# Autodesk Inventor assembly: Ensamblaje FINAL V1
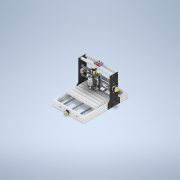
[picture p0: Inventor's stored thumbnail of the model, 180x180]
Saved by Autodesk Inventor 2021 (Build 250183000, 183)
## iProperties
Company: IMT
Created: 2022-05-28
Part Number: Ensamblaje FINAL V1
Document SubType Name: Assembly
Designer: BRAYAN GERSON DURAN TOCONAS
Project: CNC ROUTER IMT 212 P1
Author: BRAYAN GERSON DURAN TOCONAS
Title: CNC
Subject: proyecto IMT 212 P1
Comments: En esta carpeta esta todo el diseño en Inventor y calculos para la construcción de una maquina CNC fresadora para el proyecto final de la materia de diseño de maquinas. Esta CNC es capaz de desplazarse en 3 ejes. 2 por la herramienta y 1 por la base. Además de soportar el torque generador por la herramienta a la hora de gastar el material.
Revision Number: 3
## Documents named in this file (24)
- C:\Users\79449\Documents\CNC_DISENO_DE MAQUINAS\Piezas-Ensambles_Inventor\Ensamblaje FINAL V1.iam
- C:\Users\79449\Documents\CNC_DISENO_DE MAQUINAS\Piezas-Ensambles_Inventor\Primera_presentación\Ensamblaje1.iam
- C:\Users\79449\Documents\CNC_DISENO_DE MAQUINAS\Piezas-Ensambles_Inventor\Segunda_presentación\PlanchaLateral.ipt
- C:\Users\79449\Documents\CNC_DISENO_DE MAQUINAS\Piezas-Ensambles_Inventor\Segunda_presentación\V-SLOT_2020.ipt
- C:\Users\79449\Documents\CNC_DISENO_DE MAQUINAS\Piezas-Ensambles_Inventor\Segunda_presentación\SFU1605-1610\SFU1605 Assem.iam
- C:\Users\79449\Documents\CNC_DISENO_DE MAQUINAS\Piezas-Ensambles_Inventor\Segunda_presentación\Lap rap truc Y.iam
- C:\Users\79449\Documents\CNC_DISENO_DE MAQUINAS\Piezas-Ensambles_Inventor\Segunda_presentación\EjeBase v2.ipt
- C:\Users\79449\Documents\CNC_DISENO_DE MAQUINAS\Piezas-Ensambles_Inventor\Segunda_presentación\De truc Z.iam
- C:\Users\79449\Documents\CNC_DISENO_DE MAQUINAS\Piezas-Ensambles_Inventor\Segunda_presentación\ImpresionSoporte.ipt
- C:\Users\79449\Documents\CNC_DISENO_DE MAQUINAS\Piezas-Ensambles_Inventor\Segunda_presentación\Kep Truc KLF-10.ipt
- C:\Users\79449\Documents\CNC_DISENO_DE MAQUINAS\Piezas-Ensambles_Inventor\Segunda_presentación\Nema17\Assembly1.iam
- C:\Users\79449\Documents\CNC_DISENO_DE MAQUINAS\Piezas-Ensambles_Inventor\Segunda_presentación\Flexible Coupling 10-5.ipt
- C:\Users\79449\Documents\CNC_DISENO_DE MAQUINAS\Piezas-Ensambles_Inventor\Segunda_presentación\KFL003 block flange ball bearing 17 diameter shaft.ipt
- C:\Users\79449\Documents\Inventor\Content Center Files\R2021\es-ES\ANSI_ASME B18.5\ANSI_ASME B18.5 - 1_4 - 20 - 1 - 1_4-20 UNC.ipt
- C:\Users\79449\Documents\Inventor\Content Center Files\R2021\es-ES\BS 4183(1)\BS 4183 - M6(1).ipt
- C:\Users\79449\Documents\Inventor\Content Center Files\R2021\es-ES\AS 1110\AS 1110 - M4 x 25.ipt
- C:\Users\79449\Documents\Inventor\Content Center Files\R2021\es-ES\AS 1110\AS 1110 - M2,5 x 20.ipt
- C:\Users\79449\Documents\Inventor\Content Center Files\R2021\es-ES\AS 1110\AS 1110 - M2,5 x 10.ipt
- C:\Users\79449\Documents\Inventor\Content Center Files\R2021\es-ES\U 3284(2)\Unbrako. Hallowell Steel Collars. Inch Series - 0.5 x 1 x 7_16.ipt
- C:\Users\79449\Documents\Inventor\Content Center Files\R2021\es-ES\BS EN 24017\ISO 4017 - M4 x 8BS EN.ipt
- C:\Users\79449\Documents\Inventor\Content Center Files\R2021\es-ES\AS 1112 (2)\AS 1112 - M4  Tipo 5.ipt
- C:\Users\79449\Documents\Inventor\Content Center Files\R2021\es-ES\AS 1110\AS 1110 - M4 x 20.ipt
- C:\Users\79449\Documents\CNC_DISENO_DE MAQUINAS\Piezas-Ensambles_Inventor\Segunda_presentación\Arduino_CNC_Assembly.ipt
- C:\Users\79449\Documents\Inventor\Content Center Files\R2021\es-ES\AS 1112 (2)\AS 1112 - M2,5  Tipo 5.ipt
## Components (75 placed, 23 different names)
1. Ensamblaje1:1 [sub-assembly] — Nivelación:1, Coincidencia:1, Nivelación:2, Coincidencia:2, Nivelación:4, Coincidencia:23, Nivelación:13, Nivelación:14, Nivelación:15, Coincidencia:44, Coincidencia:45, Coincidencia:49, Coincidencia:50, Coincidencia:52, Coincidencia:54
2. PlanchaLateral:2 — Coincidencia:2, Nivelación:4, Coincidencia:13, Nivelación:8, Coincidencia:15, Coincidencia:19, Nivelación:11, Coincidencia:20, Nivelación:12, Nivelación:15, Coincidencia:24, Nivelación:20, Coincidencia:37, Coincidencia:39, Coincidencia:40, Coincidencia:73, Coincidencia:74, Coincidencia:75, Coincidencia:76, Coincidencia:85, Coincidencia:86, Coincidencia:87, Coincidencia:88, Coincidencia:93, Coincidencia:94, Coincidencia:113, Coincidencia:114, Coincidencia:115, Coincidencia:116, Coincidencia:117, Coincidencia:118, Coincidencia:119, Coincidencia:120, Coincidencia:121, Coincidencia:122, Coincidencia:123, Coincidencia:124, Coincidencia:125, Coincidencia:126, Coincidencia:127, Coincidencia:128, Coincidencia:130, Coincidencia:132, Coincidencia:134, Coincidencia:136, Coincidencia:138, Coincidencia:140, Coincidencia:154, Coincidencia:156, Coincidencia:158, Coincidencia:166
3. V-SLOT_2020:2 — Coincidencia:13, Coincidencia:16, Nivelación:16, Nivelación:17, Coincidencia:155, Coincidencia:159, Coincidencia:165, Nivelación:21
4. SFU1605 Assem:1 [sub-assembly] — Coincidencia:14, Coincidencia:38, Coincidencia:41, Coincidencia:43
5. Lap rap truc Y:1 [sub-assembly] — Coincidencia:14, Ángulo:1, Coincidencia:18, Coincidencia:21, Coincidencia:22, Coincidencia:27, Coincidencia:28, Coincidencia:29, Coincidencia:30
6. V-SLOT_2020:3 — Nivelación:8, Coincidencia:15, Coincidencia:16, Nivelación:19, Nivelación:20, Coincidencia:157, Coincidencia:163
7. V-SLOT_2020:4 — Coincidencia:18, Nivelación:18, Coincidencia:153, Coincidencia:161
8. EjeBase v2:1 — Coincidencia:19, Nivelación:11, Coincidencia:24, Coincidencia:25, Coincidencia:27, Coincidencia:28, Coincidencia:89, Coincidencia:91
9. EjeBase v2:2 — Coincidencia:20, Nivelación:12, Coincidencia:26, Coincidencia:29, Coincidencia:30, Coincidencia:90, Coincidencia:92
10. De truc Z:1 [sub-assembly] — Coincidencia:21, Coincidencia:22
11. PlanchaLateral:3 — Coincidencia:23, Nivelación:13, Nivelación:14, Nivelación:16, Nivelación:17, Nivelación:18, Coincidencia:25, Coincidencia:26, Nivelación:19, Coincidencia:31, Coincidencia:32, Coincidencia:33, Coincidencia:62, Coincidencia:64, Coincidencia:66, Coincidencia:68, Coincidencia:70, Coincidencia:72, Coincidencia:95, Coincidencia:96, Coincidencia:97, Coincidencia:98, Coincidencia:99, Coincidencia:100, Coincidencia:101, Coincidencia:102, Coincidencia:103, Coincidencia:104, Coincidencia:105, Coincidencia:106, Coincidencia:107, Coincidencia:108, Coincidencia:109, Coincidencia:110, Coincidencia:111, Coincidencia:112, Coincidencia:142, Coincidencia:144, Coincidencia:146, Coincidencia:148, Coincidencia:150, Coincidencia:152, Coincidencia:160, Coincidencia:162, Coincidencia:164
12. ImpresionSoporte:1 — Coincidencia:31, Coincidencia:32, Coincidencia:33, Coincidencia:34, Coincidencia:35, Coincidencia:36, Coincidencia:65, Coincidencia:67, Coincidencia:69, Coincidencia:71, Coincidencia:168, Coincidencia:170, Coincidencia:172, Coincidencia:174
13. Kep Truc KLF-10:1 — Coincidencia:34, Coincidencia:35, Coincidencia:36, Coincidencia:61, Coincidencia:63, Coincidencia:176, Coincidencia:178
14. Assembly1:1 [sub-assembly] — Coincidencia:37, Coincidencia:38, Coincidencia:39, Coincidencia:40, Coincidencia:42
15. Flexible Coupling 10-5:1 — Coincidencia:41, Coincidencia:42, Coincidencia:43
16. KFL003 block flange ball bearing 17 diameter shaft:1 — Coincidencia:44, Coincidencia:45, Coincidencia:51, Coincidencia:53, Coincidencia:58, Coincidencia:60
17. Perno de cabeza en T - Pulgadas 1/4 - 20 - 1:1 — Coincidencia:49, Coincidencia:50, Coincidencia:51, Coincidencia:57
18. Perno de cabeza en T - Pulgadas 1/4 - 20 - 1:2 — Coincidencia:52, Coincidencia:53, Coincidencia:54, Coincidencia:59
19. BS 4183 - Métrico M6:2 — Coincidencia:57, Coincidencia:58
20. BS 4183 - Métrico M6:3 — Coincidencia:59, Coincidencia:60
21. AS 1110 - Métrico M4 x 25:1 — Coincidencia:61, Coincidencia:62, Coincidencia:175
22. AS 1110 - Métrico M4 x 25:2 — Coincidencia:63, Coincidencia:64, Coincidencia:177
23. AS 1110 - Métrico M2,5 x 20:1 — Coincidencia:65, Coincidencia:66, Coincidencia:167
24. AS 1110 - Métrico M2,5 x 20:2 — Coincidencia:67, Coincidencia:68, Coincidencia:173
25. AS 1110 - Métrico M2,5 x 20:3 — Coincidencia:69, Coincidencia:70, Coincidencia:169
26. AS 1110 - Métrico M2,5 x 20:4 — Coincidencia:71, Coincidencia:72, Coincidencia:171
27. AS 1110 - Métrico M2,5 x 10:1 — Coincidencia:73, Coincidencia:74
28. AS 1110 - Métrico M2,5 x 10:2 — Coincidencia:75, Coincidencia:76
29. AS 1110 - Métrico M2,5 x 10:7 — Coincidencia:85, Coincidencia:86
30. AS 1110 - Métrico M2,5 x 10:8 — Coincidencia:87, Coincidencia:88
31. Anillo de ajuste 0.5 x 1 x 7/16:1 — Coincidencia:90, Coincidencia:96
32. Anillo de ajuste 0.5 x 1 x 7/16:2 — Coincidencia:89, Coincidencia:95
33. Anillo de ajuste 0.5 x 1 x 7/16:3 — Coincidencia:91, Coincidencia:93
34. Anillo de ajuste 0.5 x 1 x 7/16:4 — Coincidencia:92, Coincidencia:94
35. BS EN 24017 - Métrico M4 x 8:1 — Coincidencia:97, Coincidencia:98, Coincidencia:151
36. BS EN 24017 - Métrico M4 x 8:2 — Coincidencia:99, Coincidencia:100
37. BS EN 24017 - Métrico M4 x 8:3 — Coincidencia:101, Coincidencia:102
38. BS EN 24017 - Métrico M4 x 8:4 — Coincidencia:103, Coincidencia:104, Coincidencia:143
39. BS EN 24017 - Métrico M4 x 8:5 — Coincidencia:105, Coincidencia:106, Coincidencia:141
40. BS EN 24017 - Métrico M4 x 8:6 — Coincidencia:107, Coincidencia:108, Coincidencia:147
41. BS EN 24017 - Métrico M4 x 8:7 — Coincidencia:109, Coincidencia:110, Coincidencia:149
42. BS EN 24017 - Métrico M4 x 8:8 — Coincidencia:111, Coincidencia:112, Coincidencia:145
43. BS EN 24017 - Métrico M4 x 8:9 — Coincidencia:113, Coincidencia:114, Coincidencia:137
44. BS EN 24017 - Métrico M4 x 8:10 — Coincidencia:115, Coincidencia:116
45. BS EN 24017 - Métrico M4 x 8:11 — Coincidencia:117, Coincidencia:118
46. BS EN 24017 - Métrico M4 x 8:12 — Coincidencia:119, Coincidencia:120, Coincidencia:129
47. BS EN 24017 - Métrico M4 x 8:13 — Coincidencia:121, Coincidencia:122, Coincidencia:135
48. BS EN 24017 - Métrico M4 x 8:14 — Coincidencia:123, Coincidencia:124, Coincidencia:133
49. BS EN 24017 - Métrico M4 x 8:15 — Coincidencia:125, Coincidencia:126, Coincidencia:131
50. BS EN 24017 - Métrico M4 x 8:16 — Coincidencia:127, Coincidencia:128, Coincidencia:139
51. AS 1112 (2) - Métrico M4  Tipo 5:1 — Coincidencia:129, Coincidencia:130
52. AS 1112 (2) - Métrico M4  Tipo 5:2 — Coincidencia:131, Coincidencia:132
53. AS 1112 (2) - Métrico M4  Tipo 5:3 — Coincidencia:133, Coincidencia:134
54. AS 1112 (2) - Métrico M4  Tipo 5:4 — Coincidencia:135, Coincidencia:136
55. AS 1112 (2) - Métrico M4  Tipo 5:5 — Coincidencia:137, Coincidencia:138
56. AS 1112 (2) - Métrico M4  Tipo 5:6 — Coincidencia:139, Coincidencia:140
57. AS 1112 (2) - Métrico M4  Tipo 5:7 — Coincidencia:141, Coincidencia:142
58. AS 1112 (2) - Métrico M4  Tipo 5:8 — Coincidencia:143, Coincidencia:144
59. AS 1112 (2) - Métrico M4  Tipo 5:9 — Coincidencia:145, Coincidencia:146
60. AS 1112 (2) - Métrico M4  Tipo 5:10 — Coincidencia:147, Coincidencia:148
61. AS 1112 (2) - Métrico M4  Tipo 5:11 — Coincidencia:149, Coincidencia:150
62. AS 1112 (2) - Métrico M4  Tipo 5:12 — Coincidencia:151, Coincidencia:152
63. AS 1110 - Métrico M4 x 20:1 — Coincidencia:153, Coincidencia:154
64. AS 1110 - Métrico M4 x 20:2 — Coincidencia:155, Coincidencia:156
65. AS 1110 - Métrico M4 x 20:3 — Coincidencia:157, Coincidencia:158
66. AS 1110 - Métrico M4 x 20:4 — Coincidencia:159, Coincidencia:160
67. AS 1110 - Métrico M4 x 20:5 — Coincidencia:161, Coincidencia:162
68. AS 1110 - Métrico M4 x 20:6 — Coincidencia:163, Coincidencia:164
69. Arduino_CNC_Assembly:1 — Coincidencia:165, Nivelación:21, Coincidencia:166
70. AS 1112 (2) - Métrico M2,5  Tipo 5:1 — Coincidencia:167, Coincidencia:168
71. AS 1112 (2) - Métrico M2,5  Tipo 5:2 — Coincidencia:169, Coincidencia:170
72. AS 1112 (2) - Métrico M2,5  Tipo 5:3 — Coincidencia:171, Coincidencia:172
73. AS 1112 (2) - Métrico M2,5  Tipo 5:4 — Coincidencia:173, Coincidencia:174
74. AS 1112 (2) - Métrico M4  Tipo 5:13 — Coincidencia:175, Coincidencia:176
75. AS 1112 (2) - Métrico M4  Tipo 5:14 — Coincidencia:177, Coincidencia:178
## Relationships (170: Mate 154, Flush 15, Angle 1)
- Nivelación:1 [Flush]: Ensamblaje1:1
- Coincidencia:1 [Mate]: Ensamblaje1:1
- Nivelación:2 [Flush]: Ensamblaje1:1
- Coincidencia:2 [Mate]: Ensamblaje1:1 ↔ PlanchaLateral:2
- Nivelación:4 [Flush]: Ensamblaje1:1 ↔ PlanchaLateral:2
- Coincidencia:13 [Mate]: PlanchaLateral:2 ↔ V-SLOT_2020:2
- Coincidencia:14 [Mate]: SFU1605 Assem:1 ↔ Lap rap truc Y:1
- Ángulo:1 [Angle] (0 deg): Lap rap truc Y:1
- Nivelación:8 [Flush]: PlanchaLateral:2 ↔ V-SLOT_2020:3
- Coincidencia:15 [Mate]: PlanchaLateral:2 ↔ V-SLOT_2020:3
- Coincidencia:16 [Mate] (130 mm): V-SLOT_2020:2 ↔ V-SLOT_2020:3
- Coincidencia:18 [Mate]: Lap rap truc Y:1 ↔ V-SLOT_2020:4
- Coincidencia:19 [Mate]: PlanchaLateral:2 ↔ EjeBase v2:1
- Nivelación:11 [Flush]: PlanchaLateral:2 ↔ EjeBase v2:1
- Coincidencia:20 [Mate]: PlanchaLateral:2 ↔ EjeBase v2:2
- Nivelación:12 [Flush]: PlanchaLateral:2 ↔ EjeBase v2:2
- Coincidencia:21 [Mate]: Lap rap truc Y:1 ↔ De truc Z:1
- Coincidencia:22 [Mate]: Lap rap truc Y:1 ↔ De truc Z:1
- Coincidencia:23 [Mate]: Ensamblaje1:1 ↔ PlanchaLateral:3
- Nivelación:13 [Flush]: Ensamblaje1:1 ↔ PlanchaLateral:3
- Nivelación:14 [Flush] (100 mm): Ensamblaje1:1 ↔ PlanchaLateral:3
- Nivelación:15 [Flush] (-100 mm): Ensamblaje1:1 ↔ PlanchaLateral:2
- Nivelación:16 [Flush]: V-SLOT_2020:2 ↔ PlanchaLateral:3
- Nivelación:17 [Flush]: V-SLOT_2020:2 ↔ PlanchaLateral:3
- Nivelación:18 [Flush]: V-SLOT_2020:4 ↔ PlanchaLateral:3
- Coincidencia:24 [Mate]: PlanchaLateral:2 ↔ EjeBase v2:1
- Coincidencia:25 [Mate]: EjeBase v2:1 ↔ PlanchaLateral:3
- Coincidencia:26 [Mate]: EjeBase v2:2 ↔ PlanchaLateral:3
- Nivelación:19 [Flush]: V-SLOT_2020:3 ↔ PlanchaLateral:3
- Nivelación:20 [Flush]: PlanchaLateral:2 ↔ V-SLOT_2020:3
- Coincidencia:27 [Mate]: Lap rap truc Y:1 ↔ EjeBase v2:1
- Coincidencia:28 [Mate]: Lap rap truc Y:1 ↔ EjeBase v2:1
- Coincidencia:29 [Mate]: Lap rap truc Y:1 ↔ EjeBase v2:2
- Coincidencia:30 [Mate]: Lap rap truc Y:1 ↔ EjeBase v2:2
- Coincidencia:31 [Mate]: PlanchaLateral:3 ↔ ImpresionSoporte:1
- Coincidencia:32 [Mate]: PlanchaLateral:3 ↔ ImpresionSoporte:1
- Coincidencia:33 [Mate]: PlanchaLateral:3 ↔ ImpresionSoporte:1
- Coincidencia:34 [Mate]: ImpresionSoporte:1 ↔ Kep Truc KLF-10:1
- Coincidencia:35 [Mate]: ImpresionSoporte:1 ↔ Kep Truc KLF-10:1
- Coincidencia:36 [Mate]: ImpresionSoporte:1 ↔ Kep Truc KLF-10:1
- Coincidencia:37 [Mate]: PlanchaLateral:2 ↔ Assembly1:1
- Coincidencia:38 [Mate] (2 mm): SFU1605 Assem:1 ↔ Assembly1:1
- Coincidencia:39 [Mate]: PlanchaLateral:2 ↔ Assembly1:1
- Coincidencia:40 [Mate]: PlanchaLateral:2 ↔ Assembly1:1
- Coincidencia:41 [Mate]: SFU1605 Assem:1 ↔ Flexible Coupling 10-5:1
- Coincidencia:42 [Mate]: Assembly1:1 ↔ Flexible Coupling 10-5:1
- Coincidencia:43 [Mate]: SFU1605 Assem:1 ↔ Flexible Coupling 10-5:1
- Coincidencia:44 [Mate]: Ensamblaje1:1 ↔ KFL003 block flange ball bearing 17 diameter shaft:1
- Coincidencia:45 [Mate]: Ensamblaje1:1 ↔ KFL003 block flange ball bearing 17 diameter shaft:1
- Coincidencia:49 [Mate]: Ensamblaje1:1 ↔ Perno de cabeza en T - Pulgadas 1/4 - 20 - 1:1
- Coincidencia:50 [Mate]: Ensamblaje1:1 ↔ Perno de cabeza en T - Pulgadas 1/4 - 20 - 1:1
- Coincidencia:51 [Mate]: KFL003 block flange ball bearing 17 diameter shaft:1 ↔ Perno de cabeza en T - Pulgadas 1/4 - 20 - 1:1
- Coincidencia:52 [Mate]: Ensamblaje1:1 ↔ Perno de cabeza en T - Pulgadas 1/4 - 20 - 1:2
- Coincidencia:53 [Mate]: KFL003 block flange ball bearing 17 diameter shaft:1 ↔ Perno de cabeza en T - Pulgadas 1/4 - 20 - 1:2
- Coincidencia:54 [Mate]: Ensamblaje1:1 ↔ Perno de cabeza en T - Pulgadas 1/4 - 20 - 1:2
- Coincidencia:57 [Mate]: Perno de cabeza en T - Pulgadas 1/4 - 20 - 1:1 ↔ BS 4183 - Métrico M6:2
- Coincidencia:58 [Mate]: KFL003 block flange ball bearing 17 diameter shaft:1 ↔ BS 4183 - Métrico M6:2
- Coincidencia:59 [Mate]: Perno de cabeza en T - Pulgadas 1/4 - 20 - 1:2 ↔ BS 4183 - Métrico M6:3
- Coincidencia:60 [Mate]: KFL003 block flange ball bearing 17 diameter shaft:1 ↔ BS 4183 - Métrico M6:3
- Coincidencia:61 [Mate]: Kep Truc KLF-10:1 ↔ AS 1110 - Métrico M4 x 25:1
- Coincidencia:62 [Mate]: PlanchaLateral:3 ↔ AS 1110 - Métrico M4 x 25:1
- Coincidencia:63 [Mate]: Kep Truc KLF-10:1 ↔ AS 1110 - Métrico M4 x 25:2
- Coincidencia:64 [Mate]: PlanchaLateral:3 ↔ AS 1110 - Métrico M4 x 25:2
- Coincidencia:65 [Mate]: ImpresionSoporte:1 ↔ AS 1110 - Métrico M2,5 x 20:1
- Coincidencia:66 [Mate]: PlanchaLateral:3 ↔ AS 1110 - Métrico M2,5 x 20:1
- Coincidencia:67 [Mate]: ImpresionSoporte:1 ↔ AS 1110 - Métrico M2,5 x 20:2
- Coincidencia:68 [Mate]: PlanchaLateral:3 ↔ AS 1110 - Métrico M2,5 x 20:2
- Coincidencia:69 [Mate]: ImpresionSoporte:1 ↔ AS 1110 - Métrico M2,5 x 20:3
- Coincidencia:70 [Mate]: PlanchaLateral:3 ↔ AS 1110 - Métrico M2,5 x 20:3
- Coincidencia:71 [Mate]: ImpresionSoporte:1 ↔ AS 1110 - Métrico M2,5 x 20:4
- Coincidencia:72 [Mate]: PlanchaLateral:3 ↔ AS 1110 - Métrico M2,5 x 20:4
- Coincidencia:73 [Mate]: PlanchaLateral:2 ↔ AS 1110 - Métrico M2,5 x 10:1
- Coincidencia:74 [Mate]: PlanchaLateral:2 ↔ AS 1110 - Métrico M2,5 x 10:1
- Coincidencia:75 [Mate]: PlanchaLateral:2 ↔ AS 1110 - Métrico M2,5 x 10:2
- Coincidencia:76 [Mate]: PlanchaLateral:2 ↔ AS 1110 - Métrico M2,5 x 10:2
- Coincidencia:85 [Mate]: PlanchaLateral:2 ↔ AS 1110 - Métrico M2,5 x 10:7
- Coincidencia:86 [Mate]: PlanchaLateral:2 ↔ AS 1110 - Métrico M2,5 x 10:7
- Coincidencia:87 [Mate]: PlanchaLateral:2 ↔ AS 1110 - Métrico M2,5 x 10:8
- Coincidencia:88 [Mate]: PlanchaLateral:2 ↔ AS 1110 - Métrico M2,5 x 10:8
- Coincidencia:89 [Mate]: EjeBase v2:1 ↔ Anillo de ajuste 0.5 x 1 x 7/16:2
- Coincidencia:90 [Mate]: EjeBase v2:2 ↔ Anillo de ajuste 0.5 x 1 x 7/16:1
- Coincidencia:91 [Mate]: EjeBase v2:1 ↔ Anillo de ajuste 0.5 x 1 x 7/16:3
- Coincidencia:92 [Mate]: EjeBase v2:2 ↔ Anillo de ajuste 0.5 x 1 x 7/16:4
- Coincidencia:93 [Mate]: PlanchaLateral:2 ↔ Anillo de ajuste 0.5 x 1 x 7/16:3
- Coincidencia:94 [Mate]: PlanchaLateral:2 ↔ Anillo de ajuste 0.5 x 1 x 7/16:4
- Coincidencia:95 [Mate]: PlanchaLateral:3 ↔ Anillo de ajuste 0.5 x 1 x 7/16:2
- Coincidencia:96 [Mate]: PlanchaLateral:3 ↔ Anillo de ajuste 0.5 x 1 x 7/16:1
- Coincidencia:97 [Mate]: PlanchaLateral:3 ↔ BS EN 24017 - Métrico M4 x 8:1
- Coincidencia:98 [Mate]: PlanchaLateral:3 ↔ BS EN 24017 - Métrico M4 x 8:1
- Coincidencia:99 [Mate]: PlanchaLateral:3 ↔ BS EN 24017 - Métrico M4 x 8:2
- Coincidencia:100 [Mate]: PlanchaLateral:3 ↔ BS EN 24017 - Métrico M4 x 8:2
- Coincidencia:101 [Mate]: PlanchaLateral:3 ↔ BS EN 24017 - Métrico M4 x 8:3
- Coincidencia:102 [Mate]: PlanchaLateral:3 ↔ BS EN 24017 - Métrico M4 x 8:3
- Coincidencia:103 [Mate]: PlanchaLateral:3 ↔ BS EN 24017 - Métrico M4 x 8:4
- Coincidencia:104 [Mate]: PlanchaLateral:3 ↔ BS EN 24017 - Métrico M4 x 8:4
- Coincidencia:105 [Mate]: PlanchaLateral:3 ↔ BS EN 24017 - Métrico M4 x 8:5
- Coincidencia:106 [Mate]: PlanchaLateral:3 ↔ BS EN 24017 - Métrico M4 x 8:5
- Coincidencia:107 [Mate]: PlanchaLateral:3 ↔ BS EN 24017 - Métrico M4 x 8:6
- Coincidencia:108 [Mate]: PlanchaLateral:3 ↔ BS EN 24017 - Métrico M4 x 8:6
- Coincidencia:109 [Mate]: PlanchaLateral:3 ↔ BS EN 24017 - Métrico M4 x 8:7
- Coincidencia:110 [Mate]: PlanchaLateral:3 ↔ BS EN 24017 - Métrico M4 x 8:7
- Coincidencia:111 [Mate]: PlanchaLateral:3 ↔ BS EN 24017 - Métrico M4 x 8:8
- Coincidencia:112 [Mate]: PlanchaLateral:3 ↔ BS EN 24017 - Métrico M4 x 8:8
- Coincidencia:113 [Mate]: PlanchaLateral:2 ↔ BS EN 24017 - Métrico M4 x 8:9
- Coincidencia:114 [Mate]: PlanchaLateral:2 ↔ BS EN 24017 - Métrico M4 x 8:9
- Coincidencia:115 [Mate]: PlanchaLateral:2 ↔ BS EN 24017 - Métrico M4 x 8:10
- Coincidencia:116 [Mate]: PlanchaLateral:2 ↔ BS EN 24017 - Métrico M4 x 8:10
- Coincidencia:117 [Mate]: PlanchaLateral:2 ↔ BS EN 24017 - Métrico M4 x 8:11
- Coincidencia:118 [Mate]: PlanchaLateral:2 ↔ BS EN 24017 - Métrico M4 x 8:11
- Coincidencia:119 [Mate]: PlanchaLateral:2 ↔ BS EN 24017 - Métrico M4 x 8:12
- Coincidencia:120 [Mate]: PlanchaLateral:2 ↔ BS EN 24017 - Métrico M4 x 8:12
- Coincidencia:121 [Mate]: PlanchaLateral:2 ↔ BS EN 24017 - Métrico M4 x 8:13
- Coincidencia:122 [Mate]: PlanchaLateral:2 ↔ BS EN 24017 - Métrico M4 x 8:13
- Coincidencia:123 [Mate]: PlanchaLateral:2 ↔ BS EN 24017 - Métrico M4 x 8:14
- Coincidencia:124 [Mate]: PlanchaLateral:2 ↔ BS EN 24017 - Métrico M4 x 8:14
- Coincidencia:125 [Mate]: PlanchaLateral:2 ↔ BS EN 24017 - Métrico M4 x 8:15
- Coincidencia:126 [Mate]: PlanchaLateral:2 ↔ BS EN 24017 - Métrico M4 x 8:15
- Coincidencia:127 [Mate]: PlanchaLateral:2 ↔ BS EN 24017 - Métrico M4 x 8:16
- Coincidencia:128 [Mate]: PlanchaLateral:2 ↔ BS EN 24017 - Métrico M4 x 8:16
- Coincidencia:129 [Mate]: BS EN 24017 - Métrico M4 x 8:12 ↔ AS 1112 (2) - Métrico M4  Tipo 5:1
- Coincidencia:130 [Mate]: PlanchaLateral:2 ↔ AS 1112 (2) - Métrico M4  Tipo 5:1
- Coincidencia:131 [Mate]: BS EN 24017 - Métrico M4 x 8:15 ↔ AS 1112 (2) - Métrico M4  Tipo 5:2
- Coincidencia:132 [Mate]: PlanchaLateral:2 ↔ AS 1112 (2) - Métrico M4  Tipo 5:2
- Coincidencia:133 [Mate]: BS EN 24017 - Métrico M4 x 8:14 ↔ AS 1112 (2) - Métrico M4  Tipo 5:3
- Coincidencia:134 [Mate]: PlanchaLateral:2 ↔ AS 1112 (2) - Métrico M4  Tipo 5:3
- Coincidencia:135 [Mate]: BS EN 24017 - Métrico M4 x 8:13 ↔ AS 1112 (2) - Métrico M4  Tipo 5:4
- Coincidencia:136 [Mate]: PlanchaLateral:2 ↔ AS 1112 (2) - Métrico M4  Tipo 5:4
- Coincidencia:137 [Mate]: BS EN 24017 - Métrico M4 x 8:9 ↔ AS 1112 (2) - Métrico M4  Tipo 5:5
- Coincidencia:138 [Mate]: PlanchaLateral:2 ↔ AS 1112 (2) - Métrico M4  Tipo 5:5
- Coincidencia:139 [Mate]: BS EN 24017 - Métrico M4 x 8:16 ↔ AS 1112 (2) - Métrico M4  Tipo 5:6
- Coincidencia:140 [Mate]: PlanchaLateral:2 ↔ AS 1112 (2) - Métrico M4  Tipo 5:6
- Coincidencia:141 [Mate]: BS EN 24017 - Métrico M4 x 8:5 ↔ AS 1112 (2) - Métrico M4  Tipo 5:7
- Coincidencia:142 [Mate]: PlanchaLateral:3 ↔ AS 1112 (2) - Métrico M4  Tipo 5:7
- Coincidencia:143 [Mate]: BS EN 24017 - Métrico M4 x 8:4 ↔ AS 1112 (2) - Métrico M4  Tipo 5:8
- Coincidencia:144 [Mate]: PlanchaLateral:3 ↔ AS 1112 (2) - Métrico M4  Tipo 5:8
- Coincidencia:145 [Mate]: BS EN 24017 - Métrico M4 x 8:8 ↔ AS 1112 (2) - Métrico M4  Tipo 5:9
- Coincidencia:146 [Mate]: PlanchaLateral:3 ↔ AS 1112 (2) - Métrico M4  Tipo 5:9
- Coincidencia:147 [Mate]: BS EN 24017 - Métrico M4 x 8:6 ↔ AS 1112 (2) - Métrico M4  Tipo 5:10
- Coincidencia:148 [Mate]: PlanchaLateral:3 ↔ AS 1112 (2) - Métrico M4  Tipo 5:10
- Coincidencia:149 [Mate]: BS EN 24017 - Métrico M4 x 8:7 ↔ AS 1112 (2) - Métrico M4  Tipo 5:11
- Coincidencia:150 [Mate]: PlanchaLateral:3 ↔ AS 1112 (2) - Métrico M4  Tipo 5:11
- Coincidencia:151 [Mate]: BS EN 24017 - Métrico M4 x 8:1 ↔ AS 1112 (2) - Métrico M4  Tipo 5:12
- Coincidencia:152 [Mate]: PlanchaLateral:3 ↔ AS 1112 (2) - Métrico M4  Tipo 5:12
- Coincidencia:153 [Mate]: V-SLOT_2020:4 ↔ AS 1110 - Métrico M4 x 20:1
- Coincidencia:154 [Mate]: PlanchaLateral:2 ↔ AS 1110 - Métrico M4 x 20:1
- Coincidencia:155 [Mate]: V-SLOT_2020:2 ↔ AS 1110 - Métrico M4 x 20:2
- Coincidencia:156 [Mate]: PlanchaLateral:2 ↔ AS 1110 - Métrico M4 x 20:2
- Coincidencia:157 [Mate]: V-SLOT_2020:3 ↔ AS 1110 - Métrico M4 x 20:3
- Coincidencia:158 [Mate]: PlanchaLateral:2 ↔ AS 1110 - Métrico M4 x 20:3
- Coincidencia:159 [Mate]: V-SLOT_2020:2 ↔ AS 1110 - Métrico M4 x 20:4
- Coincidencia:160 [Mate]: PlanchaLateral:3 ↔ AS 1110 - Métrico M4 x 20:4
- Coincidencia:161 [Mate]: V-SLOT_2020:4 ↔ AS 1110 - Métrico M4 x 20:5
- Coincidencia:162 [Mate]: PlanchaLateral:3 ↔ AS 1110 - Métrico M4 x 20:5
- Coincidencia:163 [Mate]: V-SLOT_2020:3 ↔ AS 1110 - Métrico M4 x 20:6
- Coincidencia:164 [Mate]: PlanchaLateral:3 ↔ AS 1110 - Métrico M4 x 20:6
- Coincidencia:165 [Mate]: V-SLOT_2020:2 ↔ Arduino_CNC_Assembly:1
- Nivelación:21 [Flush] (12 mm): V-SLOT_2020:2 ↔ Arduino_CNC_Assembly:1
- Coincidencia:166 [Mate] (163 mm): PlanchaLateral:2 ↔ Arduino_CNC_Assembly:1
- Coincidencia:167 [Mate]: AS 1110 - Métrico M2,5 x 20:1 ↔ AS 1112 (2) - Métrico M2,5  Tipo 5:1
- Coincidencia:168 [Mate]: ImpresionSoporte:1 ↔ AS 1112 (2) - Métrico M2,5  Tipo 5:1
- Coincidencia:169 [Mate]: AS 1110 - Métrico M2,5 x 20:3 ↔ AS 1112 (2) - Métrico M2,5  Tipo 5:2
- Coincidencia:170 [Mate]: ImpresionSoporte:1 ↔ AS 1112 (2) - Métrico M2,5  Tipo 5:2
- Coincidencia:171 [Mate]: AS 1110 - Métrico M2,5 x 20:4 ↔ AS 1112 (2) - Métrico M2,5  Tipo 5:3
- Coincidencia:172 [Mate]: ImpresionSoporte:1 ↔ AS 1112 (2) - Métrico M2,5  Tipo 5:3
- Coincidencia:173 [Mate]: AS 1110 - Métrico M2,5 x 20:2 ↔ AS 1112 (2) - Métrico M2,5  Tipo 5:4
- Coincidencia:174 [Mate]: ImpresionSoporte:1 ↔ AS 1112 (2) - Métrico M2,5  Tipo 5:4
- Coincidencia:175 [Mate]: AS 1110 - Métrico M4 x 25:1 ↔ AS 1112 (2) - Métrico M4  Tipo 5:13
- Coincidencia:176 [Mate]: Kep Truc KLF-10:1 ↔ AS 1112 (2) - Métrico M4  Tipo 5:13
- Coincidencia:177 [Mate]: AS 1110 - Métrico M4 x 25:2 ↔ AS 1112 (2) - Métrico M4  Tipo 5:14
- Coincidencia:178 [Mate]: Kep Truc KLF-10:1 ↔ AS 1112 (2) - Métrico M4  Tipo 5:14
